# Autodesk Inventor assembly: test assembly 1
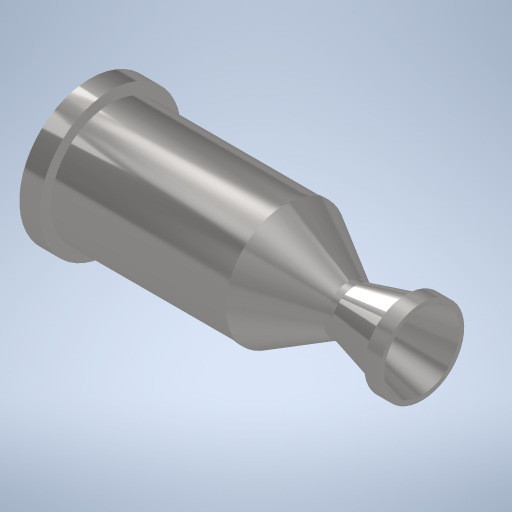
[picture p0: Inventor's stored thumbnail of the model, 512x512]
Saved by Autodesk Inventor 2023 (Build 270158000, 158)
## iProperties
Created: 2022-09-14
Part Number: test assembly 1
Document SubType Name: Assembly
Designer: station
Author: station
## Documents named in this file (3)
- C:\Users\station\Documents\Project\Liquid-engine-cooling-system\design files\ethanol engine 6\test assembly 1.iam
- C:\Users\station\Documents\Project\Liquid-engine-cooling-system\design files\ethanol engine 6\combustion chamber.ipt
- C:\Users\station\Documents\Project\Liquid-engine-cooling-system\design files\ethanol engine 6\nozzle.ipt
## Components (2 placed, 2 different names)
1. combustion chamber:1 — Mate:1, Mate:2
2. nozzle:1 — Mate:1, Mate:2
## Relationships (2: Mate 2)
- Mate:1: combustion chamber:1 ↔ nozzle:1
- Mate:2: combustion chamber:1 ↔ nozzle:1
